# Autodesk Inventor assembly: rolstoel
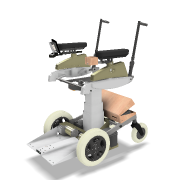
[picture p0: Inventor's stored thumbnail of the model, 180x180]
Saved by Autodesk Inventor 2020.3 (Build 243373000, 373)
## iProperties
Created: 2020-09-16
Part Number: rolstoel
Document SubType Name: Assembly
Designer: Svend
Author: Svend
## Documents named in this file (37)
- C:\Users\Svend\OneDrive\Documents\GitHub\Rolstoel\rolstoel.iam
- C:\Users\Svend\OneDrive\Documents\GitHub\Rolstoel\lift.iam
- C:\Users\Svend\OneDrive\Documents\GitHub\Rolstoel\zitvlak.iam
- C:\Users\Svend\OneDrive\Documents\GitHub\Rolstoel\onderkant.iam
- C:\Users\Svend\OneDrive\Documents\GitHub\Rolstoel\sitting_mannequin.ipt
- C:\Users\Svend\OneDrive\Documents\GitHub\Rolstoel\accu.ipt
- C:\Users\Svend\OneDrive\Documents\GitHub\Rolstoel\rplidar.iam
- C:\Users\Svend\OneDrive\Documents\GitHub\Rolstoel\IntelRealsense_D435_Multibody.ipt
- C:\Users\Svend\OneDrive\Documents\GitHub\Rolstoel\zijkant voetensteun.ipt
- C:\Users\Svend\OneDrive\Documents\GitHub\Rolstoel\voetensteun v2.ipt
- C:\Users\Svend\OneDrive\Documents\GitHub\Rolstoel\backing plate lidar.ipt
- C:\Users\Svend\OneDrive\Documents\Inventor\Content Center Files\R2020\en-US\ISO 7380-1\ISO 7380-1 - M5 x 12.ipt
- C:\Users\Svend\OneDrive\Documents\Inventor\Content Center Files\R2020\en-US\ISO 7380-1\ISO 7380-1 - M3 x 12.ipt
- C:\Users\Svend\OneDrive\Documents\Inventor\Content Center Files\R2020\en-US\ISO 7380-1\ISO 7380-1 - M4 x 12.ipt
- C:\Users\Svend\OneDrive\Documents\Inventor\Content Center Files\R2020\en-US\ISO 7380-1\ISO 7380-1 - M8 x 10.ipt
- C:\Users\Svend\OneDrive\Documents\Inventor\Content Center Files\R2020\en-US\ISO 7380-1\ISO 7380-1 - M16 x 45.ipt
- C:\Users\Svend\OneDrive\Documents\Inventor\Content Center Files\R2020\en-US\ISO 7380-1\ISO 7380-1 - M8 x 55.ipt
- C:\Users\Svend\OneDrive\Documents\Inventor\Content Center Files\R2020\en-US\ISO 7380-1\ISO 7380-1 - M10 x 40.ipt
- C:\Users\Svend\OneDrive\Documents\Inventor\Content Center Files\R2020\en-US\ISO 4161\ISO 4161 - M8(1).ipt
- C:\Users\Svend\OneDrive\Documents\Inventor\Content Center Files\R2020\en-US\ISO 10642(1)\ISO 10642 - M8x35.ipt
- C:\Users\Svend\OneDrive\Documents\Inventor\Content Center Files\R2020\en-US\ISO 4762(2)\ISO 4762 - M6 x 12ISO.ipt
- C:\Users\Svend\OneDrive\Documents\Inventor\Content Center Files\R2020\en-US\ISO 4762(2)\ISO 4762 - M6 x 10ISO.ipt
- C:\Users\Svend\OneDrive\Documents\Inventor\Content Center Files\R2020\en-US\ISO 4032(2)\ISO 4032 - M10 - ISO.ipt
- C:\Users\Svend\OneDrive\Documents\GitHub\Rolstoel\spacer electronica.ipt
- C:\Users\Svend\OneDrive\Documents\Inventor\Content Center Files\R2020\en-US\ISO 7380-1\ISO 7380-1 - M4 x 6.ipt
- C:\Users\Svend\OneDrive\Documents\GitHub\Rolstoel\elektrobox v2.iam
- C:\Users\Svend\OneDrive\Documents\GitHub\Rolstoel\module.ipt
- C:\Users\Svend\OneDrive\Documents\GitHub\Rolstoel\Raspi7inch_Case_SD_Access.ipt
- C:\Users\Svend\OneDrive\Documents\GitHub\Rolstoel\Raspi7inch_Front.ipt
- C:\Users\Svend\OneDrive\Documents\GitHub\Rolstoel\Raspi7inch_SD_Hatch.ipt
- C:\Users\Svend\OneDrive\Documents\GitHub\Rolstoel\HMI arm bewegende deel.ipt
- C:\Users\Svend\OneDrive\Documents\GitHub\Rolstoel\HMI arm vaste deel.ipt
- C:\Users\Svend\OneDrive\Documents\GitHub\Rolstoel\draaischijf HMI.ipt
- C:\Users\Svend\OneDrive\Documents\GitHub\Rolstoel\HMI achterzijde.ipt
- C:\Users\Svend\OneDrive\Documents\GitHub\Rolstoel\zijkant voetensteun rechts v2.ipt
- C:\Users\Svend\OneDrive\Documents\GitHub\Rolstoel\knoppendoosje.iam
- C:\Users\Svend\OneDrive\Documents\GitHub\Rolstoel\joystick doosje.iam
## Components (79 placed, 36 different names)
1. lift:1 [sub-assembly] — Mate:1, Mate:2, Mate:3, Mate:4, Mate:5, Mate:6, Mate:7, Mate:8, Flush:1, Flush:9
2. zitvlak:1 [sub-assembly] — Mate:1, Mate:2, Mate:3, Flush:2, Flush:3, Flush:4, Mate:37, Mate:38, Mate:39, Mate:40, Insert:34, Insert:35, Insert:36, Insert:37, Insert:46, Insert:47, Insert:48, Insert:50, Mate:61, Mate:62, Mate:63, Mate:68, Mate:69, Mate:70, Angle:64, Mate:71, Mate:72, Flush:68
3. onderkant:1 [sub-assembly] — Mate:4, Mate:5, Mate:6, Mate:9, Mate:10, Mate:11, Mate:12, Mate:13, Mate:14, Mate:20, Mate:31, Insert:32, Insert:33, Mate:41, Mate:42, Insert:38, Insert:39, Insert:40, Insert:41, Insert:42, Insert:43, Insert:44, Insert:45, Mate:44, Mate:45, Mate:46, Mate:47, Mate:48, Flush:50, Flush:51, Flush:63, Flush:65, Flush:66, Flush:67
4. sitting_mannequin:1 — Flush:2, Flush:3, Flush:4
5. accu:1 — Mate:9, Mate:10, Mate:11
6. accu:2 — Mate:12, Mate:13, Mate:14
7. rplidar:1 [sub-assembly] — Mate:26, Mate:25, Mate:27
8. IntelRealsense_D435_Multibody:1 — Mate:26, Mate:23, Flush:8, Mate:28
9. zijkant voetensteun:1 — Mate:20, Flush:10, Mate:67, Flush:63, Flush:67
10. voetensteun v2:1 — Mate:23, Flush:8, Mate:25, Mate:27, Mate:28, Flush:9, Flush:10, Mate:34, Mate:35, Mate:36, Insert:1, Insert:2, Insert:3, Insert:4, Insert:5, Insert:6, Insert:7, Mate:67
11. zijkant voetensteun rechts v2:1 — Mate:31, Flush:65, Flush:66
12. backing plate lidar:1 — Mate:34, Mate:35, Mate:36
13. ISO 7380-1 M5 x 12:1 — Insert:1
14. ISO 7380-1 M3 x 12:1 — Insert:2
15. ISO 7380-1 M3 x 12:2 — Insert:3
16. ISO 7380-1 M3 x 12:3 — Insert:4
17. ISO 7380-1 M3 x 12:4 — Insert:5
18. ISO 7380-1 M4 x 12:1 — Insert:6
19. ISO 7380-1 M4 x 12:2 — Insert:7
20. ISO 7380-1 M4 x 12:3
21. ISO 7380-1 M4 x 12:4
22. ISO 7380-1 M4 x 12:5
23. ISO 7380-1 M4 x 12:6
24. ISO 7380-1 M4 x 12:7
25. ISO 7380-1 M4 x 12:8
26. ISO 7380-1 M4 x 12:9
27. ISO 7380-1 M4 x 12:10
28. ISO 7380-1 M4 x 12:11
29. ISO 7380-1 M4 x 12:12
30. ISO 7380-1 M4 x 12:13
31. ISO 7380-1 M4 x 12:18
32. ISO 7380-1 M8 x 10:1
33. ISO 7380-1 M8 x 10:2
34. ISO 7380-1 M8 x 10:3
35. ISO 7380-1 M8 x 10:4
36. ISO 7380-1 M8 x 10:5
37. ISO 7380-1 M8 x 10:6
38. ISO 7380-1 M8 x 10:7
39. ISO 7380-1 M8 x 10:8
40. ISO 7380-1 M16 x 45:1 — Insert:32
41. ISO 7380-1 M16 x 45:2 — Insert:33
42. ISO 7380-1 M8 x 55:1 — Mate:37, Mate:38
43. ISO 7380-1 M8 x 55:2 — Mate:39, Mate:40
44. ISO 7380-1 M10 x 40:1 — Insert:34
45. ISO 7380-1 M10 x 40:2 — Insert:35
46. ISO 4161 M8:1 — Insert:36
47. ISO 4161 M8:2 — Insert:37
48. ISO 10642 M8x35:1 — Mate:41
49. ISO 10642 M8x35:2 — Mate:42
50. ISO 4762 M6 x 12:1 — Insert:38
51. ISO 4762 M6 x 12:2 — Insert:39
52. ISO 4762 M6 x 12:3 — Insert:40
53. ISO 4762 M6 x 12:4 — Insert:41
54. ISO 4762 M6 x 10:1 — Insert:42
55. ISO 4762 M6 x 10:2 — Insert:43
56. ISO 4762 M6 x 10:3 — Insert:44
57. ISO 4762 M6 x 10:4 — Insert:45
58. ISO 4161 M8:3 — Insert:46
59. ISO 4161 M8:4 — Insert:47
60. ISO 4032 M10:1 — Insert:48, Insert:49
61. ISO 4032 M10:2 — Insert:49
62. ISO 4032 M10:3 — Insert:50
63. spacer electronica:1 — Mate:46, Mate:47
64. ISO 7380-1 M4 x 6:1
65. ISO 7380-1 M4 x 6:2
66. ISO 7380-1 M4 x 6:3
67. ISO 7380-1 M4 x 6:4
68. spacer electronica:2 — Mate:44, Mate:45
69. elektrobox v2:1 [sub-assembly] — Mate:48, Flush:50, Flush:51
70. module:1 — Mate:53, Flush:54, Flush:55
71. Raspi7inch_Case_SD_Access:1 — Mate:54, Flush:56, Flush:57, Mate:55, Flush:58, Mate:56, Flush:60, Flush:61, Flush:62
72. Raspi7inch_Front:1 — Mate:53, Flush:54, Flush:55, Mate:54, Flush:56, Flush:57
73. Raspi7inch_SD_Hatch:1 — Mate:55, Flush:58, Mate:56
74. HMI arm bewegende deel:1 — Mate:57, Mate:58, Mate:59, Mate:60
75. HMI arm vaste deel:1 — Mate:59, Mate:60, Mate:61, Mate:62, Mate:63, Angle:63
76. draaischijf HMI:1 — Mate:57, Mate:58, Mate:64, Mate:65, Angle:63, Mate:66
77. HMI achterzijde:1 — Flush:60, Mate:64, Mate:65, Flush:61, Flush:62, Mate:66
78. knoppendoosje:1 [sub-assembly] — Mate:68, Mate:69, Mate:70, Angle:64
79. joystick doosje:1 [sub-assembly] — Mate:71, Mate:72, Flush:68
## Relationships (105: Mate 55, Insert 26, Flush 22, Angle 2)
- Mate:1: lift:1 ↔ zitvlak:1
- Mate:2: lift:1 ↔ zitvlak:1
- Mate:3: lift:1 ↔ zitvlak:1
- Mate:4: lift:1 ↔ onderkant:1
- Mate:5: lift:1 ↔ onderkant:1
- Mate:6 (10 mm): lift:1 ↔ onderkant:1
- Mate:7: lift:1
- Mate:8: lift:1
- Flush:1: lift:1
- Flush:2: zitvlak:1 ↔ sitting_mannequin:1
- Flush:3 (-300 mm): zitvlak:1 ↔ sitting_mannequin:1
- Flush:4 (50 mm): zitvlak:1 ↔ sitting_mannequin:1
- Mate:9: onderkant:1 ↔ accu:1
- Mate:10 (10 mm): onderkant:1 ↔ accu:1
- Mate:11 (2 mm): onderkant:1 ↔ accu:1
- Mate:12: onderkant:1 ↔ accu:2
- Mate:13 (10 mm): onderkant:1 ↔ accu:2
- Mate:14 (2 mm): onderkant:1 ↔ accu:2
- Mate:20: onderkant:1 ↔ zijkant voetensteun:1
- Mate:26: rplidar:1 ↔ IntelRealsense_D435_Multibody:1
- Mate:23: IntelRealsense_D435_Multibody:1 ↔ voetensteun v2:1
- Flush:8: IntelRealsense_D435_Multibody:1 ↔ voetensteun v2:1
- Mate:25 (4 mm): rplidar:1 ↔ voetensteun v2:1
- Mate:27 (-70 mm): rplidar:1 ↔ voetensteun v2:1
- Mate:28: IntelRealsense_D435_Multibody:1 ↔ voetensteun v2:1
- Flush:9: lift:1 ↔ voetensteun v2:1
- Flush:10: zijkant voetensteun:1 ↔ voetensteun v2:1
- Mate:31: onderkant:1 ↔ zijkant voetensteun rechts v2:1
- Mate:34: voetensteun v2:1 ↔ backing plate lidar:1
- Mate:35: voetensteun v2:1 ↔ backing plate lidar:1
- Mate:36 (260 mm): voetensteun v2:1 ↔ backing plate lidar:1
- Insert:1: voetensteun v2:1 ↔ ISO 7380-1 M5 x 12:1
- Insert:2: voetensteun v2:1 ↔ ISO 7380-1 M3 x 12:1
- Insert:3: voetensteun v2:1 ↔ ISO 7380-1 M3 x 12:2
- Insert:4: voetensteun v2:1 ↔ ISO 7380-1 M3 x 12:3
- Insert:5: voetensteun v2:1 ↔ ISO 7380-1 M3 x 12:4
- Insert:6: voetensteun v2:1 ↔ ISO 7380-1 M4 x 12:1
- Insert:7: voetensteun v2:1 ↔ ISO 7380-1 M4 x 12:2
- Insert:32: onderkant:1 ↔ ISO 7380-1 M16 x 45:1
- Insert:33: onderkant:1 ↔ ISO 7380-1 M16 x 45:2
- Mate:37: zitvlak:1 ↔ ISO 7380-1 M8 x 55:1
- Mate:38: zitvlak:1 ↔ ISO 7380-1 M8 x 55:1
- Mate:39: zitvlak:1 ↔ ISO 7380-1 M8 x 55:2
- Mate:40: zitvlak:1 ↔ ISO 7380-1 M8 x 55:2
- Insert:34: zitvlak:1 ↔ ISO 7380-1 M10 x 40:1
- Insert:35: zitvlak:1 ↔ ISO 7380-1 M10 x 40:2
- Insert:36: zitvlak:1 ↔ ISO 4161 M8:1
- Insert:37: zitvlak:1 ↔ ISO 4161 M8:2
- Mate:41: onderkant:1 ↔ ISO 10642 M8x35:1
- Mate:42: onderkant:1 ↔ ISO 10642 M8x35:2
- Insert:38: onderkant:1 ↔ ISO 4762 M6 x 12:1
- Insert:39: onderkant:1 ↔ ISO 4762 M6 x 12:2
- Insert:40: onderkant:1 ↔ ISO 4762 M6 x 12:3
- Insert:41: onderkant:1 ↔ ISO 4762 M6 x 12:4
- Insert:42: onderkant:1 ↔ ISO 4762 M6 x 10:1
- Insert:43: onderkant:1 ↔ ISO 4762 M6 x 10:2
- Insert:44: onderkant:1 ↔ ISO 4762 M6 x 10:3
- Insert:45: onderkant:1 ↔ ISO 4762 M6 x 10:4
- Insert:46: zitvlak:1 ↔ ISO 4161 M8:3
- Insert:47: zitvlak:1 ↔ ISO 4161 M8:4
- Insert:48: zitvlak:1 ↔ ISO 4032 M10:1
- Insert:49: ISO 4032 M10:1 ↔ ISO 4032 M10:2
- Insert:50: zitvlak:1 ↔ ISO 4032 M10:3
- Mate:44: onderkant:1 ↔ spacer electronica:2
- Mate:45: onderkant:1 ↔ spacer electronica:2
- Mate:46: onderkant:1 ↔ spacer electronica:1
- Mate:47: onderkant:1 ↔ spacer electronica:1
- Mate:48: onderkant:1 ↔ elektrobox v2:1
- Flush:50: onderkant:1 ↔ elektrobox v2:1
- Flush:51: onderkant:1 ↔ elektrobox v2:1
- Mate:53: module:1 ↔ Raspi7inch_Front:1
- Flush:54: module:1 ↔ Raspi7inch_Front:1
- Flush:55: module:1 ↔ Raspi7inch_Front:1
- Mate:54: Raspi7inch_Case_SD_Access:1 ↔ Raspi7inch_Front:1
- Flush:56 (27.7 mm): Raspi7inch_Case_SD_Access:1 ↔ Raspi7inch_Front:1
- Flush:57 (10.4 mm): Raspi7inch_Case_SD_Access:1 ↔ Raspi7inch_Front:1
- Mate:55: Raspi7inch_Case_SD_Access:1 ↔ Raspi7inch_SD_Hatch:1
- Flush:58: Raspi7inch_Case_SD_Access:1 ↔ Raspi7inch_SD_Hatch:1
- Mate:56: Raspi7inch_Case_SD_Access:1 ↔ Raspi7inch_SD_Hatch:1
- Mate:57: HMI arm bewegende deel:1 ↔ draaischijf HMI:1
- Mate:58: HMI arm bewegende deel:1 ↔ draaischijf HMI:1
- Mate:59: HMI arm bewegende deel:1 ↔ HMI arm vaste deel:1
- Mate:60: HMI arm bewegende deel:1 ↔ HMI arm vaste deel:1
- Mate:61 (0.5 mm): zitvlak:1 ↔ HMI arm vaste deel:1
- Mate:62 (0.5 mm): zitvlak:1 ↔ HMI arm vaste deel:1
- Mate:63: zitvlak:1 ↔ HMI arm vaste deel:1
- Flush:60: Raspi7inch_Case_SD_Access:1 ↔ HMI achterzijde:1
- Mate:64: draaischijf HMI:1 ↔ HMI achterzijde:1
- Mate:65: draaischijf HMI:1 ↔ HMI achterzijde:1
- Flush:61: Raspi7inch_Case_SD_Access:1 ↔ HMI achterzijde:1
- Flush:62: Raspi7inch_Case_SD_Access:1 ↔ HMI achterzijde:1
- Angle:63 (0 deg): HMI arm vaste deel:1 ↔ draaischijf HMI:1
- Mate:66: draaischijf HMI:1 ↔ HMI achterzijde:1
- Mate:67: zijkant voetensteun:1 ↔ voetensteun v2:1
- Flush:63: onderkant:1 ↔ zijkant voetensteun:1
- Flush:65: onderkant:1 ↔ zijkant voetensteun rechts v2:1
- Flush:66: onderkant:1 ↔ zijkant voetensteun rechts v2:1
- Flush:67: onderkant:1 ↔ zijkant voetensteun:1
- Mate:68: zitvlak:1 ↔ knoppendoosje:1
- Mate:69 (-30 mm): zitvlak:1 ↔ knoppendoosje:1
- Mate:70: zitvlak:1 ↔ knoppendoosje:1
- Angle:64 (0 deg): zitvlak:1 ↔ knoppendoosje:1
- Mate:71: zitvlak:1 ↔ joystick doosje:1
- Mate:72: zitvlak:1 ↔ joystick doosje:1
- Flush:68: zitvlak:1 ↔ joystick doosje:1
